# Autodesk Inventor assembly: 7 Pin Male
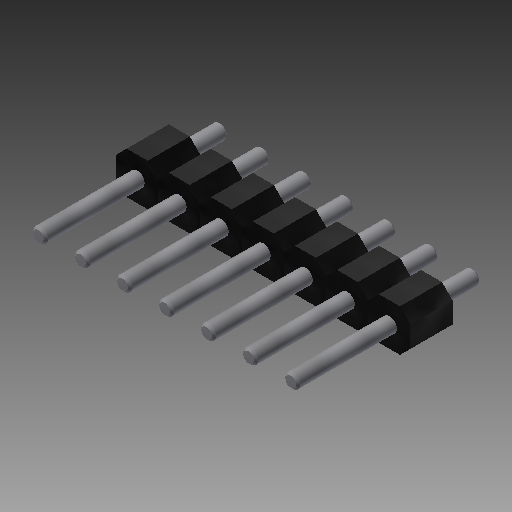
[picture p0: Inventor's stored thumbnail of the model, 512x512]
Saved by Autodesk Inventor 2017 (Build 210142000, 142)
## iProperties
Created: 2016-08-05
Part Number: 7 Pin Male
Document SubType Name: Assembly
Designer: ge937963
Author: ge937963
## Documents named in this file (2)
- Z:\allusers\Diagnostics\Inventor Files\3dPrintedPCR\7 Pin Male.iam
- Z:\allusers\Diagnostics\Inventor Files\3dPrintedPCR\Pin.ipt
## Components (7 placed, 1 different names)
1. Pin:1 — Flush:1, Flush:7, Mate:1
2. Pin:2 — Flush:1, Flush:2, Flush:7, Flush:8, Mate:1, Mate:2
3. Pin:3 — Flush:2, Flush:3, Flush:8, Flush:9, Mate:2, Mate:3
4. Pin:4 — Flush:3, Flush:4, Flush:9, Flush:10, Mate:3, Mate:4
5. Pin:5 — Flush:4, Flush:5, Flush:10, Flush:11, Mate:4, Mate:5
6. Pin:6 — Flush:5, Flush:6, Flush:11, Flush:12, Mate:5, Mate:6
7. Pin:7 — Flush:6, Flush:12, Mate:6
## Relationships (18: Flush 12, Mate 6)
- Flush:1: Pin:1 ↔ Pin:2
- Flush:2: Pin:2 ↔ Pin:3
- Flush:3: Pin:3 ↔ Pin:4
- Flush:4: Pin:4 ↔ Pin:5
- Flush:5: Pin:5 ↔ Pin:6
- Flush:6: Pin:6 ↔ Pin:7
- Flush:7: Pin:1 ↔ Pin:2
- Flush:8: Pin:2 ↔ Pin:3
- Flush:9: Pin:3 ↔ Pin:4
- Flush:10: Pin:4 ↔ Pin:5
- Flush:11: Pin:5 ↔ Pin:6
- Flush:12: Pin:6 ↔ Pin:7
- Mate:1: Pin:1 ↔ Pin:2
- Mate:2: Pin:2 ↔ Pin:3
- Mate:3: Pin:3 ↔ Pin:4
- Mate:4: Pin:4 ↔ Pin:5
- Mate:5: Pin:5 ↔ Pin:6
- Mate:6: Pin:6 ↔ Pin:7
